# Autodesk Inventor assembly: Assembly_V7
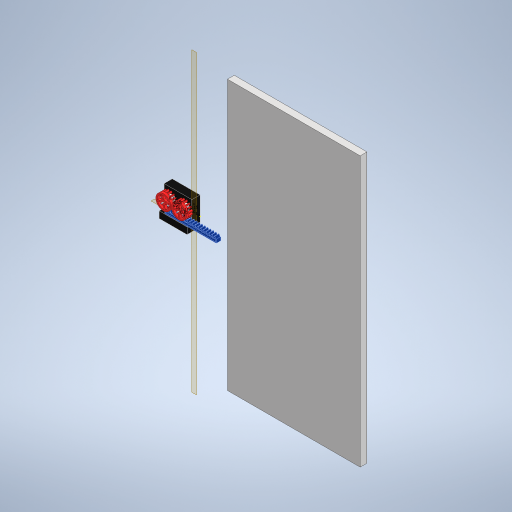
[picture p0: Inventor's stored thumbnail of the model, 512x512]
Saved by Autodesk Inventor 2023 (Build 270158000, 158)
## iProperties
Created: 2023-03-29
Part Number: Assembly_V7
Document SubType Name: Assembly
Designer: shrey
Author: shrey
## Documents named in this file (12)
- D:\Inventor Projects\Door Lock\V7\Assembly_V7.iam
- D:\Inventor Projects\Door Lock\V4\moulding.ipt
- D:\Inventor Projects\Door Lock\motor.ipt
- D:\Inventor Projects\Door Lock\V6\pinion_nohole_V6.ipt
- D:\Inventor Projects\Door Lock\V6\pinion_V6.ipt
- D:\Inventor Projects\Door Lock\V7\mountingPlate_V7.ipt
- D:\Inventor Projects\Door Lock\V7\rack_V7.ipt
- D:\Inventor Projects\Door Lock\V7\Assembly_V7\Design Accelerator\Spur Gears1.iam
- D:\Inventor Projects\Door Lock\V7\pinion_V7.ipt
- D:\Inventor Projects\Door Lock\V6\ESP-12F.ipt
- D:\Inventor Projects\Door Lock\V7\door.ipt
- D:\Inventor Projects\Door Lock\L293D_PowerDIP16_Package.ipt
## Components (13 placed, 11 different names)
1. moulding:1 — Mate:1, Flush:1, Flush:2, Mate:7, Mate:13, Mate:14, Flush:16, Mate:23, Mate:24, Flush:21
2. motor:1 — Mate:4, Mate:6, Flush:3, Flush:13, Flush:15, Mate:13, Mate:17, Mate:18, Mate:20
3. pinion_nohole_V6:1 — Mate:4, Mate:5
4. motor:2 — Mate:2, Mate:3, Mate:6, Flush:3, Mate:7, Mate:15, Mate:16, Mate:19, Mate:20
5. pinion_V6:1 — Mate:2, Mate:3, Mate:5
6. mountingPlate_V7:1 — Mate:9, Mate:10, Flush:4, Flush:16, Flush:17, Flush:18, Flush:19, Flush:20, Flush:22, Mate:26
7. rack_V7:1 — Flush:13, Flush:14, Flush:15, Mate:14
8. Spur Gears:1 [sub-assembly]
9. pinion_V7:1 — Mate:15, Mate:16, Mate:19
10. pinion_V7:2 — Mate:17, Mate:18
11. ESP-12F:1 — Flush:17, Flush:18, Flush:19, Flush:20, Flush:23
12. door:1 — Mate:22, Mate:23, Mate:24, Flush:21
13. L293D — Flush:22, Mate:26, Flush:23
## Relationships (36: Mate 21, Flush 15)
- Mate:1: moulding:1
- Flush:1: moulding:1
- Flush:2: moulding:1
- Mate:2: motor:2 ↔ pinion_V6:1
- Mate:3: motor:2 ↔ pinion_V6:1
- Mate:4: motor:1 ↔ pinion_nohole_V6:1
- Mate:5 (1 mm): pinion_nohole_V6:1 ↔ pinion_V6:1
- Mate:6: motor:1 ↔ motor:2
- Flush:3: motor:1 ↔ motor:2
- Mate:7 (14 mm): moulding:1 ↔ motor:2
- Mate:9: mountingPlate_V7:1
- Mate:10: mountingPlate_V7:1
- Flush:4: mountingPlate_V7:1
- Flush:13 (2.5 mm): motor:1 ↔ rack_V7:1
- Flush:14: rack_V7:1
- Flush:15 (14 mm): motor:1 ↔ rack_V7:1
- Mate:13 (1 mm): moulding:1 ↔ motor:1
- Mate:14: moulding:1 ↔ rack_V7:1
- Mate:15: motor:2 ↔ pinion_V7:1
- Mate:16: motor:2 ↔ pinion_V7:1
- Mate:17: motor:1 ↔ pinion_V7:2
- Mate:18: motor:1 ↔ pinion_V7:2
- Mate:19: motor:2 ↔ pinion_V7:1
- Mate:20 (-35 mm): motor:1 ↔ motor:2
- Flush:16: moulding:1 ↔ mountingPlate_V7:1
- Flush:17: mountingPlate_V7:1 ↔ ESP-12F:1
- Flush:18 (2 mm): mountingPlate_V7:1 ↔ ESP-12F:1
- Flush:19 (5 mm): mountingPlate_V7:1 ↔ ESP-12F:1
- Flush:20: mountingPlate_V7:1 ↔ ESP-12F:1
- Mate:22: door:1
- Mate:23: moulding:1 ↔ door:1
- Mate:24: moulding:1 ↔ door:1
- Flush:21: moulding:1 ↔ door:1
- Flush:22 (5 mm): mountingPlate_V7:1 ↔ L293D
- Mate:26 (-9 mm): mountingPlate_V7:1 ↔ L293D
- Flush:23: ESP-12F:1 ↔ L293D
